# Autodesk Inventor assembly: actuator
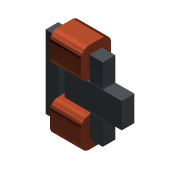
[picture p0: Inventor's stored thumbnail of the model, 180x180]
Saved by Autodesk Inventor 2018.2 (Build 222227000, 227)
## iProperties
Created: 2019-02-04
Part Number: actuator
Document SubType Name: Assembly
Designer: ns6022
Author: ns6022
## Documents named in this file (4)
- C:\GoogleDrive\Teaching\Courses\Industrial_Electronics_2_EENG27000\EM_Lab\EM_model\actuator.iam
- C:\GoogleDrive\Teaching\Courses\Industrial_Electronics_2_EENG27000\EM_Lab\EM_model\Core.ipt
- C:\GoogleDrive\Teaching\Courses\Industrial_Electronics_2_EENG27000\EM_Lab\EM_model\Armature.ipt
- C:\GoogleDrive\Teaching\Courses\Industrial_Electronics_2_EENG27000\EM_Lab\EM_model\Winding.ipt
## Components (4 placed, 3 different names)
1. Core:1 — Flush:1, Mate:1, Mate:2, Mate:3, Mate:4, Mate:5, Mate:6, Mate:7, Mate:8
2. Armature:1 — Flush:1, Mate:1, Mate:2
3. Winding:1 — Mate:3, Mate:4, Mate:5
4. Winding:2 — Mate:6, Mate:7, Mate:8
## Relationships (9: Mate 8, Flush 1)
- Flush:1: Core:1 ↔ Armature:1
- Mate:1 (10 mm): Core:1 ↔ Armature:1
- Mate:2 (0.5 mm): Core:1 ↔ Armature:1
- Mate:3 (0.5 mm): Core:1 ↔ Winding:1
- Mate:4 (0.5 mm): Core:1 ↔ Winding:1
- Mate:5 (0.5 mm): Core:1 ↔ Winding:1
- Mate:6 (0.5 mm): Core:1 ↔ Winding:2
- Mate:7 (0.5 mm): Core:1 ↔ Winding:2
- Mate:8 (0.5 mm): Core:1 ↔ Winding:2
